# Autodesk Inventor assembly: roscas
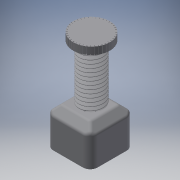
[picture p0: Inventor's stored thumbnail of the model, 180x180]
Saved by Autodesk Inventor 2019 (Build 230136000, 136)
## iProperties
Created: 2018-12-22
Part Number: roscas
Document SubType Name: Assembly
Designer: assman
Author: assman
## Documents named in this file (3)
- D:\Inventor\CatFeeder\tests\roscas.iam
- D:\Inventor\CatFeeder\tests\rosca_hembra.ipt
- D:\Inventor\CatFeeder\tests\rosca_macho.ipt
## Components (2 placed, 2 different names)
1. rosca_hembra:1 — Flush:1
2. rosca_macho:1 — Flush:1
## Relationships (1: Flush 1)
- Flush:1: rosca_hembra:1 ↔ rosca_macho:1
